# Autodesk Inventor assembly: Intrepid
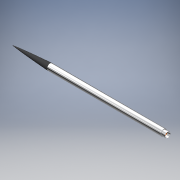
[picture p0: Inventor's stored thumbnail of the model, 180x180]
Saved by Autodesk Inventor 2017 SP1 (Build 210196100, 196)
## iProperties
Created: 2016-10-21
Part Number: Intrepid
Document SubType Name: Assembly
Designer: cflannery
Author: cflannery
## Documents named in this file (4)
- D:\Triton_Rocket_Club\NONGIT\Vehicles\Intrepid\Intrepid.iam
- D:\Triton_Rocket_Club\NONGIT\Vehicles\Intrepid\Structures\airframe.ipt
- D:\Triton_Rocket_Club\NONGIT\Vehicles\Intrepid\Structures\nosecone_0.75.ipt
- D:\Triton_Rocket_Club\NONGIT\Vehicles\Intrepid\Structures\motor.iam
## Components (3 placed, 3 different names)
1. airframe:1 — Mate:1, Mate:2, Mate:3, Flush:1
2. nosecone_0.75:1 — Mate:1, Mate:2
3. motor:1 [sub-assembly] — Mate:3, Flush:1
## Relationships (4: Mate 3, Flush 1)
- Mate:1: airframe:1 ↔ nosecone_0.75:1
- Mate:2: airframe:1 ↔ nosecone_0.75:1
- Mate:3: airframe:1 ↔ motor:1
- Flush:1: airframe:1 ↔ motor:1
